# Autodesk Inventor assembly: Aliuminium Profile Door
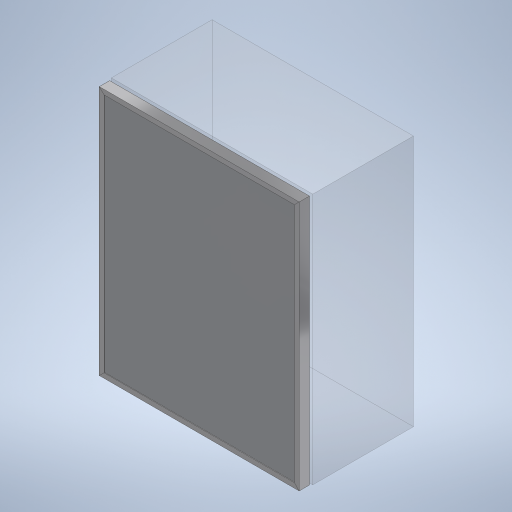
[picture p0: Inventor's stored thumbnail of the model, 512x512]
Saved by Autodesk Inventor 2024 (Build 280153000, 153)
## iProperties
RuleStatus: InUse
Created: 2014-12-01
Part Number: Aliuminium Profile Door
Document SubType Name: Assembly
Designer: SauliusD
Author: SauliusD
## Documents named in this file (7)
- C:\W4INV 2024 Design\iBOX LIBRARY\Facades\Aluminium Profile\Aliuminium Profile Door.iam
- C:\W4INV 2024 Design\iBOX LIBRARY\Facades\Aluminium Profile\Top Frame.ipt
- C:\W4INV 2024 Design\iBOX LIBRARY\Facades\Aluminium Profile\Right Frame.ipt
- C:\W4INV 2024 Design\iBOX LIBRARY\Facades\Aluminium Profile\Bottom Frame.ipt
- C:\W4INV 2024 Design\iBOX LIBRARY\Facades\Aluminium Profile\Left Frame.ipt
- C:\W4INV 2024 Design\iBOX LIBRARY\Facades\Aluminium Profile\Aliuminium Profile Door.ipt
- C:\W4INV 2024 Design\iBOX LIBRARY\Facades\Aluminium Profile\Glass_2.ipt
## Components (6 placed, 6 different names)
1. @Skeleton — Flush:1, Flush:2, Flush:3
2. Top Frame:1
3. Right Frame:1
4. Bottom Frame:1
5. Left Frame:1
6. Glass_2:1
## Relationships (3: Flush 3)
- Flush:1: @Skeleton
- Flush:2: @Skeleton
- Flush:3: @Skeleton
## Named parameters: Off_From_Left = 1.5 mm, Off_From_Right = 1.5 mm, Off_From_Top = 1.5 mm, Off_From_Bottom = 1.5 mm
